# Autodesk Inventor assembly: DHT_sestava
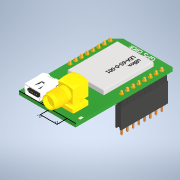
[picture p0: Inventor's stored thumbnail of the model, 180x180]
Saved by Autodesk Inventor 2022 (Build 260153000, 153)
## iProperties
Created: 2022-03-19
Part Number: DHT_sestava
Document SubType Name: Assembly
Designer: dvorakj
Author: dvorakj
## Documents named in this file (7)
- C:\Users\dvorakj\Documents\Inventor\Bakalarka\Clicks\GPS\GPS_sestava.iam
- C:\Users\dvorakj\Documents\Inventor\Bakalarka\Clicks\Pin Header\61300811121 (rev1).iam
- C:\Users\dvorakj\Documents\Inventor\Bakalarka\Clicks\tRF\SMA\SMA ANGLED.ipt
- C:\Users\dvorakj\Documents\Inventor\Bakalarka\Clicks\GPS\GPS_PCB.ipt
- C:\Users\dvorakj\Documents\Inventor\Bakalarka\Clicks\GPS\GPS.ipt
- C:\Users\dvorakj\Documents\Inventor\Bakalarka\Clicks\GPS\USB\Mini_USB.ipt
- C:\Users\dvorakj\Documents\Inventor\Bakalarka\Clicks\GPS\LED\STP_WL-SMCW_150060xx75020 (rev1).iam
## Components (8 placed, 6 different names)
1. 61300811121 (rev1):1 [sub-assembly] — Mate:3
2. 61300811121 (rev1):2 [sub-assembly] — Mate:1, Mate:2
3. SMA ANGLED:1 — Flush:1, Mate:4, Mate:5
4. GPS_PCB:1 — Mate:1, Mate:2, Mate:3, Flush:1, Mate:4, Mate:5, Flush:2, Mate:6, Flush:3, Flush:4, Flush:5, Mate:7, Mate:8, Flush:6
5. GPS:1 — Flush:2, Flush:6
6. Mini_USB:1 — Mate:6, Flush:3, Flush:4
7. STP_WL-SMCW_150060xx75020 (rev1):1 [sub-assembly] — Flush:5, Mate:8
8. STP_WL-SMCW_150060xx75020 (rev1):2 [sub-assembly] — Mate:7
## Relationships (14: Mate 8, Flush 6)
- Mate:1: 61300811121 (rev1):2 ↔ GPS_PCB:1
- Mate:2: 61300811121 (rev1):2 ↔ GPS_PCB:1
- Mate:3: 61300811121 (rev1):1 ↔ GPS_PCB:1
- Flush:1 (-4 mm): SMA ANGLED:1 ↔ GPS_PCB:1
- Mate:4 (-10 mm): SMA ANGLED:1 ↔ GPS_PCB:1
- Mate:5: SMA ANGLED:1 ↔ GPS_PCB:1
- Flush:2: GPS_PCB:1 ↔ GPS:1
- Mate:6: GPS_PCB:1 ↔ Mini_USB:1
- Flush:3 (2 mm): GPS_PCB:1 ↔ Mini_USB:1
- Flush:4: GPS_PCB:1 ↔ Mini_USB:1
- Flush:5 (13 mm): GPS_PCB:1 ↔ STP_WL-SMCW_150060xx75020 (rev1):1
- Mate:7: GPS_PCB:1 ↔ STP_WL-SMCW_150060xx75020 (rev1):2
- Mate:8: GPS_PCB:1 ↔ STP_WL-SMCW_150060xx75020 (rev1):1
- Flush:6: GPS_PCB:1 ↔ GPS:1
